# Autodesk Inventor assembly: MechSwitch_Assem_V3
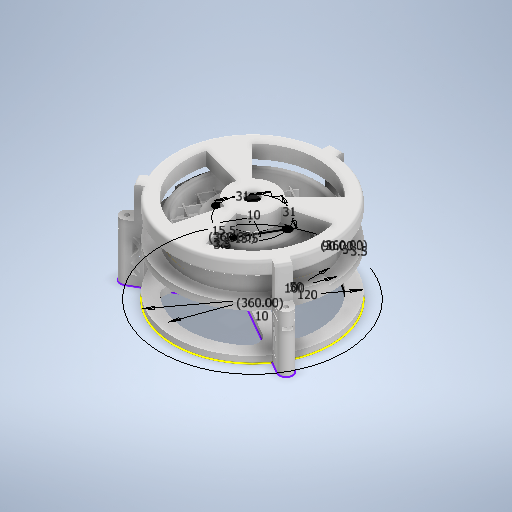
[picture p0: Inventor's stored thumbnail of the model, 512x512]
Saved by Autodesk Inventor 2025.1 (Build 291241000, 241)
## iProperties
Created: 2026-04-16
Part Number: MechSwitch_Assem_V3
Document SubType Name: Assembly
Designer: ryand
Author: ryand
## Documents named in this file (4)
- C:\Users\ryand\OneDrive\Documents\Inventor\TNG\Rotational_TENG\MechSwitch\MechSwitch_Assem_V3.iam
- C:\Users\ryand\OneDrive\Documents\Inventor\TNG\Rotational_TENG\MechSwitch\MechSwitch_MotorBaseiptV3.ipt
- C:\Users\ryand\OneDrive\Documents\Inventor\TNG\Rotational_TENG\MechSwitch\Bottom_Stand.ipt
- C:\Users\ryand\OneDrive\Documents\Inventor\TNG\Rotational_TENG\MechSwitch\MechSwitch_DielecTopV3.ipt
## Components (3 placed, 3 different names)
1. MechSwitch_MotorBaseiptV3:1 — Mate:1, Mate:2, Mate:3, Mate:4, Mate:5
2. Bottom_Stand:1 — Mate:1, Mate:2
3. MechSwitch_DielecTopV3:1 — Mate:3, Mate:4, Mate:5
## Relationships (5: Mate 5)
- Mate:1: MechSwitch_MotorBaseiptV3:1 ↔ Bottom_Stand:1
- Mate:2: MechSwitch_MotorBaseiptV3:1 ↔ Bottom_Stand:1
- Mate:3: MechSwitch_MotorBaseiptV3:1 ↔ MechSwitch_DielecTopV3:1
- Mate:4: MechSwitch_MotorBaseiptV3:1 ↔ MechSwitch_DielecTopV3:1
- Mate:5: MechSwitch_MotorBaseiptV3:1 ↔ MechSwitch_DielecTopV3:1
